# Autodesk Inventor assembly: ControllerAssembly
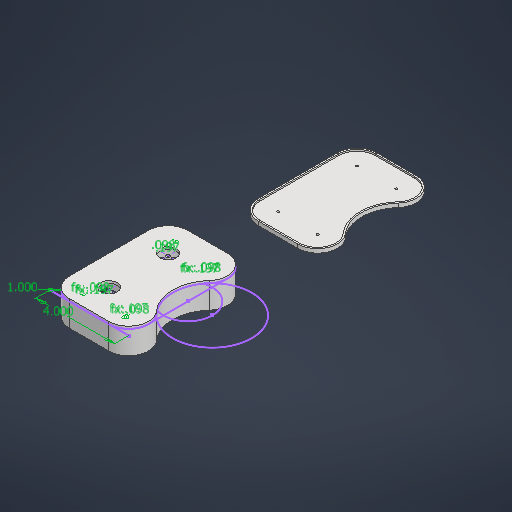
[picture p0: Inventor's stored thumbnail of the model, 512x512]
Saved by Autodesk Inventor 2026.1 (Build 301233000, 233)
## iProperties
Created: 2026-07-06
Part Number: ControllerAssembly
Document SubType Name: Assembly
Designer: Kasi Pusuluri
Author: Kasi Pusuluri
## Documents named in this file (6)
- C:\Users\Kasi Pusuluri\Documents\Outpost 2026\Controller\ControllerAssembly.iam
- C:\Users\Kasi Pusuluri\Documents\Outpost 2026\Controller\ControllerTop.ipt
- C:\Users\Kasi Pusuluri\Documents\Outpost 2026\Controller\ControllerBottom.ipt
- C:\Users\Kasi Pusuluri\Documents\Outpost 2026\BumperCarV2\PCB2.ipt
- C:\Users\Kasi Pusuluri\Documents\Outpost 2026\Controller\BatteryHolder.ipt
- C:\Users\Kasi Pusuluri\Documents\Outpost 2026\BumperCarV2\NRF24L01+.ipt
## Components (5 placed, 5 different names)
1. ControllerTop:1 — Rigid:1, Mate:1, Mate:2
2. ControllerBottom:1
3. PCB2:1 — Mate:1
4. BatteryHolder:1 — Rigid:1
5. NRF24L01+:1 — Mate:2
## Relationships (3: Mate 2, WeldJoint 1)
- Rigid:1 [WeldJoint]: ControllerTop:1 ↔ BatteryHolder:1
- Mate:1: ControllerTop:1 ↔ PCB2:1
- Mate:2: ControllerTop:1 ↔ NRF24L01+:1
